# Autodesk Inventor assembly: Spoolholder
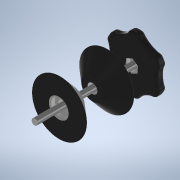
[picture p0: Inventor's stored thumbnail of the model, 180x180]
Saved by Autodesk Inventor 2020.2 (Build 242310000, 310)
## iProperties
Created: 2020-08-25
Part Number: Spoolholder
Document SubType Name: Assembly
Designer: JK
Author: JK
## Documents named in this file (4)
- C:\Users\JK\Documents\Inventor\Anet Upgrade\Spoolholder.iam
- C:\Users\JK\Documents\Inventor\Anet Upgrade\threadedrod.ipt
- C:\Users\JK\Documents\Inventor\Anet Upgrade\Cono 1.ipt
- C:\Users\JK\Documents\Inventor\Anet Upgrade\Bloqueo.ipt
## Components (4 placed, 3 different names)
1. threadedrod:1 — Mate:1, Mate:2, Mate:3
2. Cono 1:1 — Mate:2
3. Cono 1:2 — Mate:1
4. Bloqueo:1 — Mate:3
## Relationships (3: Mate 3)
- Mate:1: threadedrod:1 ↔ Cono 1:2
- Mate:2: threadedrod:1 ↔ Cono 1:1
- Mate:3: threadedrod:1 ↔ Bloqueo:1
